# Autodesk Inventor assembly: FW102C_partsremoved
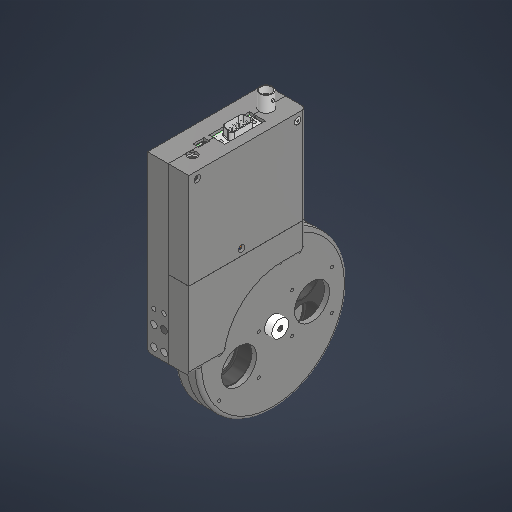
[picture p0: Inventor's stored thumbnail of the model, 512x512]
Saved by Autodesk Inventor 2026 (Build 300175050, 175E)
## iProperties
Company: Thorlabs, Inc.
Created: 2011-03-10
Part Number: FW102C_partsremoved
Description: STEP AP214
Document SubType Name: Assembly
Designer: Julian
Sending System: SolidWorks 2011
Preprocessor: SwSTEP 2.0
Title: 20242-E01.STEP
Author: Admin
Revision Number: ANY
## Documents named in this file (14)
- G:\Projects\Setup\setup_inventor_2025\filter wheel moto\FW102C_partsremoved.iam
- G:\Projects\Setup\setup_inventor_2025\filter wheel moto\OptoSensorBoard.iam
- G:\Projects\Setup\setup_inventor_2025\filter wheel moto\MainBoard.iam
- G:\Projects\Setup\setup_inventor_2025\filter wheel moto\20242-004_Engraving.ipt
- G:\Projects\Setup\setup_inventor_2025\filter wheel moto\NRPN052MAMP-RC.ipt
- G:\Projects\Setup\setup_inventor_2025\filter wheel moto\EG1526.ipt
- G:\Projects\Setup\setup_inventor_2025\filter wheel moto\20242-016.ipt
- G:\Projects\Setup\setup_inventor_2025\filter wheel moto\20242-014.ipt
- G:\Projects\Setup\setup_inventor_2025\filter wheel moto\SFWR3ST.ipt
- G:\Projects\Setup\setup_inventor_2025\filter wheel moto\20242-005.ipt
- G:\Projects\Setup\setup_inventor_2025\filter wheel moto\Socket Countersunk Head Cap Screw_AI_SCHCSCREW 0.086-56x0.25x0.25-HX-N.ipt
- G:\Projects\Setup\setup_inventor_2025\filter wheel moto\20242-017.ipt
- G:\Projects\Setup\setup_inventor_2025\filter wheel moto\98704A320.ipt
- G:\Projects\Setup\setup_inventor_2025\filter wheel moto\Wheel_FW102CWheel.iam
## Components (13 placed, 13 different names)
1. OptoSensorBoard_18 [sub-assembly]
2. MainBoard_19 [sub-assembly]
3. 20242-004_Engraving_21
4. NRPN052MAMP-RC_24
5. EG1526_27
6. 20242-016_28
7. 20242-014_29
8. SFWR3ST_30
9. 20242-005_32
10. 20242-017_35 — Tangent:1, Tangent:2
11. 98704A320_36
12. Socket Countersunk Head Cap Screw_AI_SCHCSCREW 0.086-56x0.25x0.25-HX-N_37
13. Wheel_FW102CWheel_43 [sub-assembly] — Tangent:1, Tangent:2
## Relationships (2: Tangent 2)
- Tangent:1: 20242-017_35 ↔ Wheel_FW102CWheel_43
- Tangent:2: 20242-017_35 ↔ Wheel_FW102CWheel_43
